# Autodesk Inventor assembly: power-distribution-assembly
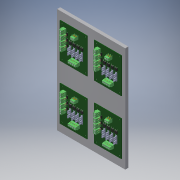
[picture p0: Inventor's stored thumbnail of the model, 180x180]
Saved by Autodesk Inventor 2019.2 (Build 232265000, 265)
## iProperties
Created: 2020-05-06
Part Number: power-distribution-assembly
Document SubType Name: Assembly
Designer: Johansson
Author: Johansson
## Documents named in this file (3)
- D:\Dropbox\Dokument\Projekt\Elita\Electrical system\Highside-Powerdistribution\hardware\cad\power-distribution-assembly.iam
- D:\Dropbox\Dokument\Projekt\Elita\Electrical system\Highside-Powerdistribution\hardware\cad\power-distribution.iam
- D:\Dropbox\Dokument\Projekt\Elita\Electrical system\Highside-Powerdistribution\hardware\cad\Fastener.ipt
## Components (5 placed, 2 different names)
1. power-distribution:1 [sub-assembly] — Insert:1, Insert:2
2. Fastener:1 — Insert:1, Insert:2, Insert:3, Insert:4, Insert:5, Insert:6, Insert:7, Insert:8
3. power-distribution:2 [sub-assembly] — Insert:3, Insert:4
4. power-distribution:3 [sub-assembly] — Insert:5, Insert:6
5. power-distribution:4 [sub-assembly] — Insert:7, Insert:8
## Relationships (8: Insert 8)
- Insert:1: power-distribution:1 ↔ Fastener:1
- Insert:2: power-distribution:1 ↔ Fastener:1
- Insert:3: Fastener:1 ↔ power-distribution:2
- Insert:4: Fastener:1 ↔ power-distribution:2
- Insert:5: Fastener:1 ↔ power-distribution:3
- Insert:6: Fastener:1 ↔ power-distribution:3
- Insert:7: Fastener:1 ↔ power-distribution:4
- Insert:8: Fastener:1 ↔ power-distribution:4
